# Autodesk Inventor assembly: mesa
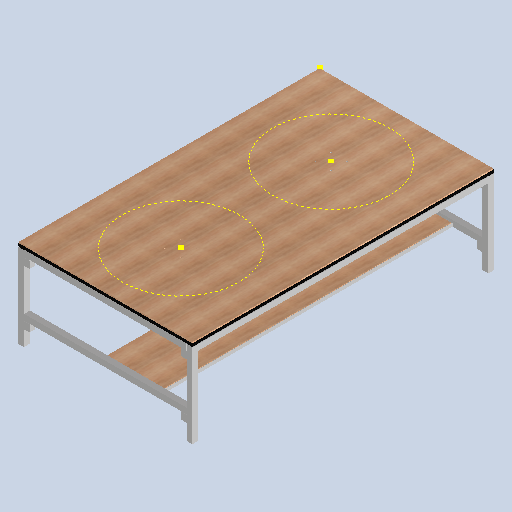
[picture p0: Inventor's stored thumbnail of the model, 512x512]
Saved by Autodesk Inventor 2025 (Build 290162000, 162)
## iProperties
Created: 2022-08-16
Part Number: mesa
Document SubType Name: Assembly
Designer: cvss2
Author: cvss2
## Documents named in this file (7)
- C:\Users\cvss2.CINSOFTEX\Documents\GitHub\general-3d-models\Robos\Denso VS050\sala\mesa2Denso\mesa2DensoVS050.iam
- C:\Users\cvss2.CINSOFTEX\Documents\GitHub\general-3d-models\Robos\Denso VS050\sala\mesa2Denso\madeiraMesa.ipt
- C:\Users\cvss2.CINSOFTEX\Documents\GitHub\general-3d-models\Robos\Denso VS050\sala\mesa2Denso\estruturaMesa.ipt
- C:\Users\cvss2.CINSOFTEX\Documents\GitHub\general-3d-models\Robos\Denso VS050\sala\mesa2Denso\PernasMesa.ipt
- C:\Users\cvss2.CINSOFTEX\Documents\GitHub\general-3d-models\Robos\Denso VS050\sala\mesa2Denso\apoioLateral.ipt
- C:\Users\cvss2.CINSOFTEX\Documents\GitHub\general-3d-models\Robos\Denso VS050\sala\mesa2Denso\apoioControladora.ipt
- C:\Users\cvss2.CINSOFTEX\Documents\GitHub\general-3d-models\Robos\Denso VS050\sala\mesa2Denso\madeiraControladora.ipt
## Components (8 placed, 6 different names)
1. madeiraMesa:1 — Mate:4, Mate:5, Mate:6
2. estruturaMesa:1 — Mate:1, Mate:2, Mate:3, Mate:4, Mate:5, Mate:6, Mate:11, Mate:12, Mate:13
3. PernasMesa:1 — Mate:1, Mate:2, Mate:3, Flush:1, Mate:7, Mate:8, Mate:19
4. PernasMesa:2 — Mate:11, Mate:12, Mate:13, Mate:14, Mate:15
5. apoioLateral:1 — Flush:1, Mate:7, Mate:8
6. apoioLateral:2
7. apoioControladora:1 — Mate:14, Mate:15, Mate:16, Mate:17, Mate:18, Mate:19
8. madeiraControladora:1 — Mate:16, Mate:17, Mate:18
## Relationships (21: Mate 19, Flush 2)
- Mate:1: estruturaMesa:1 ↔ PernasMesa:1
- Mate:2: estruturaMesa:1 ↔ PernasMesa:1
- Mate:3 (5 mm): estruturaMesa:1 ↔ PernasMesa:1
- Mate:4: madeiraMesa:1 ↔ estruturaMesa:1
- Mate:5: madeiraMesa:1 ↔ estruturaMesa:1
- Mate:6: madeiraMesa:1 ↔ estruturaMesa:1
- Flush:1: PernasMesa:1 ↔ apoioLateral:1
- Mate:7: PernasMesa:1 ↔ apoioLateral:1
- Mate:8: PernasMesa:1 ↔ apoioLateral:1
- [Flush]: PernasMesa:2 ↔ apoioLateral:2
- [Mate]: PernasMesa:2 ↔ apoioLateral:2
- [Mate]: PernasMesa:2 ↔ apoioLateral:2
- Mate:11: estruturaMesa:1 ↔ PernasMesa:2
- Mate:12: estruturaMesa:1 ↔ PernasMesa:2
- Mate:13 (5 mm): estruturaMesa:1 ↔ PernasMesa:2
- Mate:14 (2 mm): PernasMesa:2 ↔ apoioControladora:1
- Mate:15 (2 mm): PernasMesa:2 ↔ apoioControladora:1
- Mate:16: apoioControladora:1 ↔ madeiraControladora:1
- Mate:17: apoioControladora:1 ↔ madeiraControladora:1
- Mate:18: apoioControladora:1 ↔ madeiraControladora:1
- Mate:19 (3 mm): PernasMesa:1 ↔ apoioControladora:1
## Named parameters: d12_d9 = 0 mm, d13_d10 = 0 mm, d14_d11 = 0 mm, largura = 1800 mm, comprimento = 1900 mm
